# Autodesk Inventor assembly: tachobasura
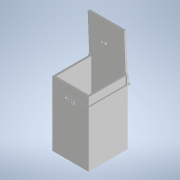
[picture p0: Inventor's stored thumbnail of the model, 180x180]
Saved by Autodesk Inventor 2021 (Build 250183000, 183)
## iProperties
Created: 2022-02-10
Part Number: tachobasura
Document SubType Name: Assembly
Designer: Emanuel
Author: Emanuel
## Documents named in this file (4)
- D:\Respaldo 4-4-2021\Desktop\ESPOL\tachobasura.iam
- D:\Respaldo 4-4-2021\Desktop\ESPOL\tacho.ipt
- D:\Respaldo 4-4-2021\Desktop\ESPOL\tapa.ipt
- D:\Respaldo 4-4-2021\Desktop\ESPOL\SENSORultimo.ipt
## Components (4 placed, 3 different names)
1. tacho:1 — De rotación:1, Coincidencia:1
2. tapa:1 — De rotación:1, Coincidencia:2
3. SENSORultimo:1 — Coincidencia:1
4. SENSORultimo:2 — Coincidencia:2
## Relationships (3: Mate 2, RevoluteJoint 1)
- De rotación:1 [RevoluteJoint]: tacho:1 ↔ tapa:1
- Coincidencia:1 [Mate]: tacho:1 ↔ SENSORultimo:1
- Coincidencia:2 [Mate]: tapa:1 ↔ SENSORultimo:2
